# Autodesk Inventor assembly: Assembly2
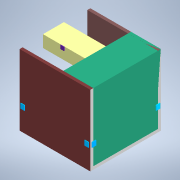
[picture p0: Inventor's stored thumbnail of the model, 180x180]
Saved by Autodesk Inventor 2022.3 (Build 263350000, 350)
## iProperties
Created: 2023-02-06
Part Number: Assembly2
Document SubType Name: Assembly
Designer: lbmcgill42
Author: lbmcgill42
## Documents named in this file (20)
- \\labdrive.tntech.edu\labdrive\lbmcgill42\Documents\Capstone Stuff\Chassis Blocks\Assembly2.iam
- \\labdrive.tntech.edu\labdrive\lbmcgill42\Documents\Capstone Stuff\Chassis Blocks\power_supply.ipt
- \\labdrive.tntech.edu\labdrive\lbmcgill42\Documents\Capstone Stuff\Chassis Blocks\Chips.ipt
- \\labdrive.tntech.edu\labdrive\lbmcgill42\Documents\Capstone Stuff\Chassis Blocks\Pedestal.ipt
- \\labdrive.tntech.edu\labdrive\lbmcgill42\Documents\Capstone Stuff\Chassis Blocks\Intake.ipt
- \\labdrive.tntech.edu\labdrive\lbmcgill42\Documents\Capstone Stuff\Chassis Blocks\Sorting.ipt
- \\labdrive.tntech.edu\labdrive\lbmcgill42\Documents\Capstone Stuff\Chassis Blocks\Jetson.ipt
- \\labdrive.tntech.edu\labdrive\lbmcgill42\Documents\Capstone Stuff\Chassis Blocks\Aduino.ipt
- \\labdrive.tntech.edu\labdrive\lbmcgill42\Documents\Capstone Stuff\Chassis Blocks\Arduino2.ipt
- \\labdrive.tntech.edu\labdrive\lbmcgill42\Documents\Capstone Stuff\Chassis Blocks\chassisFloor.ipt
- \\labdrive.tntech.edu\labdrive\lbmcgill42\Documents\ToF Sensor.ipt
- \\labdrive.tntech.edu\labdrive\lbmcgill42\Documents\ToF Sensor2.ipt
- \\labdrive.tntech.edu\labdrive\lbmcgill42\Documents\ToF Sensor3.ipt
- \\labdrive.tntech.edu\labdrive\lbmcgill42\Documents\ToF Sensor4.ipt
- \\labdrive.tntech.edu\labdrive\lbmcgill42\Documents\ToF Sensor5.ipt
- \\labdrive.tntech.edu\labdrive\lbmcgill42\Documents\ToF Sensor6.ipt
- \\labdrive.tntech.edu\labdrive\lbmcgill42\Documents\ToF Sensor7.ipt
- \\labdrive.tntech.edu\labdrive\lbmcgill42\Documents\ToF Sensor8.ipt
- \\labdrive.tntech.edu\labdrive\lbmcgill42\Documents\ColorSensor1.ipt
- \\labdrive.tntech.edu\labdrive\lbmcgill42\Documents\ColorSensor2.ipt
## Components (19 placed, 19 different names)
1. power_supply:1 — Mate:16, Flush:3, Mate:17
2. Chips:1 — Mate:5, Mate:6, Mate:7
3. Pedestal:1 — Mate:10, Mate:11, Mate:12
4. Intake:1 — Mate:7, Mate:8, Mate:9, Mate:12, Mate:13, Mate:14, Mate:16, Mate:22, Mate:23, Flush:13
5. Sorting:1 — Mate:13, Mate:14, Mate:15, Flush:3, Mate:29, Flush:23, Flush:24
6. Jetson:1 — Mate:18, Mate:19, Flush:4
7. Aduino1:1 — Mate:2, Mate:3, Mate:4, Flush:1, Flush:2
8. Arduino2:1 — Mate:2, Flush:1, Flush:2
9. chassisFloor:1 — Mate:3, Mate:4, Mate:5, Mate:6, Mate:8, Mate:9, Mate:10, Mate:11, Mate:15, Mate:17, Mate:18, Mate:19, Flush:4, Mate:20, Flush:5, Flush:6, Mate:21, Flush:7, Flush:8, Flush:9, Flush:10, Flush:11, Flush:12, Mate:24, Mate:25, Flush:14, Flush:15, Flush:16, Mate:26, Mate:27, Flush:17, Flush:18, Flush:19, Flush:20, Mate:28, Flush:21, Flush:22
10. ToF Sensor1:1 — Mate:23, Flush:11, Flush:12
11. ToF Sensor2:1 — Mate:20, Flush:5, Flush:6
12. ToF Sensor3:1 — Mate:26, Flush:17, Flush:18
13. ToF Sensor4:1 — Mate:27, Flush:19, Flush:20
14. ToF Sensor5:1 — Mate:22, Flush:9, Flush:10
15. ToF Sensor6:1 — Mate:24, Flush:13, Flush:14
16. ToF Sensor7:1 — Mate:25, Flush:15, Flush:16
17. ToF Sensor8:1 — Mate:21, Flush:7, Flush:8
18. ColorSensor1:1 — Mate:29, Flush:23, Flush:24
19. ColorSensor2:1 — Mate:28, Flush:21, Flush:22
## Relationships (52: Mate 28, Flush 24)
- Mate:2 (5.08 mm): Aduino1:1 ↔ Arduino2:1
- Mate:3 (13.97 mm): Aduino1:1 ↔ chassisFloor:1
- Mate:4: Aduino1:1 ↔ chassisFloor:1
- Flush:1: Aduino1:1 ↔ Arduino2:1
- Flush:2: Aduino1:1 ↔ Arduino2:1
- Mate:5: Chips:1 ↔ chassisFloor:1
- Mate:6: Chips:1 ↔ chassisFloor:1
- Mate:7: Chips:1 ↔ Intake:1
- Mate:8: Intake:1 ↔ chassisFloor:1
- Mate:9: Intake:1 ↔ chassisFloor:1
- Mate:10: Pedestal:1 ↔ chassisFloor:1
- Mate:11: Pedestal:1 ↔ chassisFloor:1
- Mate:12: Pedestal:1 ↔ Intake:1
- Mate:13: Intake:1 ↔ Sorting:1
- Mate:14: Intake:1 ↔ Sorting:1
- Mate:15 (93.98 mm): Sorting:1 ↔ chassisFloor:1
- Mate:16: power_supply:1 ↔ Intake:1
- Flush:3: power_supply:1 ↔ Sorting:1
- Mate:17: power_supply:1 ↔ chassisFloor:1
- Mate:18: Jetson:1 ↔ chassisFloor:1
- Mate:19: Jetson:1 ↔ chassisFloor:1
- Flush:4: Jetson:1 ↔ chassisFloor:1
- Mate:20: chassisFloor:1 ↔ ToF Sensor2:1
- Flush:5 (5.08 mm): chassisFloor:1 ↔ ToF Sensor2:1
- Flush:6 (85.09 mm): chassisFloor:1 ↔ ToF Sensor2:1
- Mate:21: chassisFloor:1 ↔ ToF Sensor8:1
- Flush:7 (5.08 mm): chassisFloor:1 ↔ ToF Sensor8:1
- Flush:8 (85.09 mm): chassisFloor:1 ↔ ToF Sensor8:1
- Mate:22: Intake:1 ↔ ToF Sensor5:1
- Mate:23: Intake:1 ↔ ToF Sensor1:1
- Flush:9 (5.08 mm): chassisFloor:1 ↔ ToF Sensor5:1
- Flush:10 (85.09 mm): chassisFloor:1 ↔ ToF Sensor5:1
- Flush:11 (5.08 mm): chassisFloor:1 ↔ ToF Sensor1:1
- Flush:12 (85.09 mm): chassisFloor:1 ↔ ToF Sensor1:1
- Mate:24: chassisFloor:1 ↔ ToF Sensor6:1
- Mate:25: chassisFloor:1 ↔ ToF Sensor7:1
- Flush:13 (5.08 mm): Intake:1 ↔ ToF Sensor6:1
- Flush:14 (85.09 mm): chassisFloor:1 ↔ ToF Sensor6:1
- Flush:15 (5.08 mm): chassisFloor:1 ↔ ToF Sensor7:1
- Flush:16 (85.09 mm): chassisFloor:1 ↔ ToF Sensor7:1
- Mate:26: chassisFloor:1 ↔ ToF Sensor3:1
- Mate:27: chassisFloor:1 ↔ ToF Sensor4:1
- Flush:17 (5.08 mm): chassisFloor:1 ↔ ToF Sensor3:1
- Flush:18 (85.09 mm): chassisFloor:1 ↔ ToF Sensor3:1
- Flush:19 (5.08 mm): chassisFloor:1 ↔ ToF Sensor4:1
- Flush:20 (85.09 mm): chassisFloor:1 ↔ ToF Sensor4:1
- Mate:28: chassisFloor:1 ↔ ColorSensor2:1
- Flush:21 (142.24 mm): chassisFloor:1 ↔ ColorSensor2:1
- Flush:22 (142.24 mm): chassisFloor:1 ↔ ColorSensor2:1
- Mate:29: Sorting:1 ↔ ColorSensor1:1
- Flush:23 (76.2 mm): Sorting:1 ↔ ColorSensor1:1
- Flush:24: Sorting:1 ↔ ColorSensor1:1
